# Autodesk Inventor assembly: blocker
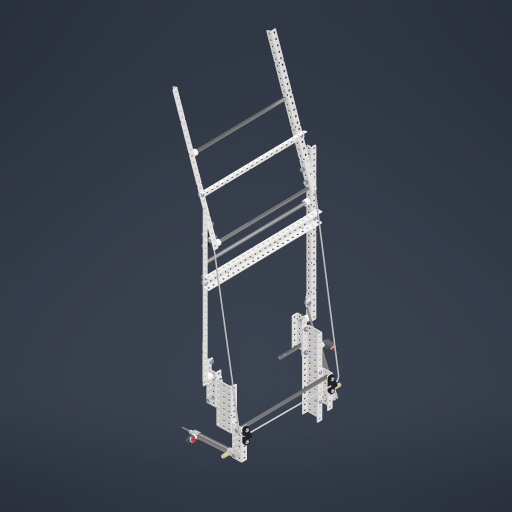
[picture p0: Inventor's stored thumbnail of the model, 512x512]
Saved by Autodesk Inventor 2024 (Build 280153000, 153)
## iProperties
Created: 2024-01-04
Part Number: blocker
Document SubType Name: Assembly
Designer: macbook
Author: macbook
## Documents named in this file (39)
- \\Mac\Home\Desktop\code\1599V-VRC\Cad\Assembly\v4\blocker.iam
- \\Mac\Home\Desktop\code\1599V-VRC\Cad\Assembly\v4\puncher.iam
- \\Mac\Home\Desktop\code\1599V-VRC\Cad\Structure\C Channel\Aluminum 1x3x1\Alu C 1x3x1x15.ipt
- \\Mac\Home\Desktop\code\1599V-VRC\Cad\Structure\C Channel\Aluminum 1x2x1\Alu C 1x2x1x6.ipt
- \\Mac\Home\Desktop\code\1599V-VRC\Cad\Motion\Pneumatics\Double Acting Piston.iam
- \\Mac\Home\Desktop\code\1599V-VRC\Cad\Structure\Standoff\Standoff 2.00.ipt
- \\Mac\Home\Desktop\code\1599V-VRC\Cad\Structure\Standoff.ipt
- \\Mac\Home\Desktop\code\1599V-VRC\Cad\Structure\C Channel\Aluminum 1x3x1\Alu C 1x3x1x8.ipt
- \\Mac\Home\Desktop\code\1599V-VRC\Cad\Structure\Standoff\Standoff 3.00.ipt
- \\Mac\Home\Desktop\code\1599V-VRC\Cad\Structure\Standoff\Standoff 6.00.ipt
- \\Mac\Home\Desktop\code\1599V-VRC\Cad\Motion\Spacers\Spacer Nylon .313 OD\NSpacer .313 OD x .125.ipt
- \\Mac\Home\Desktop\code\1599V-VRC\Cad\Motion\Spacers\Spacer Nylon .313 OD.ipt
- \\Mac\Home\Desktop\code\1599V-VRC\Cad\Structure\Angle\Aluminum\1x1\Alu Angle 1x1x30.ipt
- \\Mac\Home\Desktop\code\1599V-VRC\Cad\Motion\Spacers\Washer Teflon\TWasher .375 OD x .06250.ipt
- \\Mac\Home\Desktop\code\1599V-VRC\Cad\Motion\Spacers\Washer Teflon.ipt
- \\Mac\Home\Desktop\code\1599V-VRC\Cad\Structure\Angle\Aluminum\1x1\Alu Angle 1x1x1.ipt
- \\Mac\Home\Desktop\code\1599V-VRC\Cad\Structure\Hardware\Nut Nylock.ipt
- \\Mac\Home\Desktop\code\1599V-VRC\Cad\Structure\Angle\Aluminum\1x1\Alu Angle 1x1x25.ipt
- \\Mac\Home\Desktop\code\1599V-VRC\Cad\Motion\Shaft LS\Bearing Flat.ipt
- \\Mac\Home\Desktop\code\1599V-VRC\Cad\Structure\Hardware\Screw Steel - Star\SScrew Star Smooth .500.ipt
- \\Mac\Home\Desktop\code\1599V-VRC\Cad\Structure\Hardware\Screw Steel - Star.ipt
- \\Mac\Home\Desktop\code\1599V-VRC\Cad\Structure\Hardware\Nut Keps.ipt
- \\Mac\Home\Desktop\code\1599V-VRC\Cad\Motion\Shaft HS\HS Pillow Bearing Block.ipt
- \\Mac\Home\Desktop\code\1599V-VRC\Cad\Structure\Hardware\Screw Steel - Star\SScrew Star Smooth .375.ipt
- \\Mac\Home\Desktop\code\1599V-VRC\Cad\Motion\Pneumatics\Fitting for Cylinders.ipt
- \\Mac\Home\Desktop\code\1599V-VRC\Cad\Motion\Spacers\Spacer Nylon .500 OD\NSpacer White .500 OD x .500.ipt
- \\Mac\Home\Desktop\code\1599V-VRC\Cad\Motion\Spacers\Spacer Nylon .500 OD.ipt
- \\Mac\Home\Desktop\code\1599V-VRC\Cad\Structure\Hardware\Screw Steel - Star\SScrew Star Smooth .290.ipt
- \\Mac\Home\Desktop\code\1599V-VRC\Cad\Structure\Hardware\Screw Steel - Star\SScrew Star Smooth .875.ipt
- \\Mac\Home\Desktop\code\1599V-VRC\Cad\Motion\Insert Circle.ipt
- \\Mac\Home\Desktop\code\1599V-VRC\Cad\Structure\C Channel\Aluminum 1x2x1\Alu C 1x2x1x23.ipt
- \\Mac\Home\Desktop\code\1599V-VRC\Cad\Motion\Spacers\Spacer Nylon .313 OD\NSpacer .313 OD x .375.ipt
- \\Mac\Home\Desktop\code\1599V-VRC\Cad\Motion\Spacers\Spacer Nylon .500 OD\NSpacer White .500 OD x .375.ipt
- \\Mac\Home\Desktop\code\1599V-VRC\Cad\Structure\Angle\Aluminum\1x1\Alu Angle 1x1x21.ipt
- \\Mac\Home\Desktop\code\1599V-VRC\Cad\Structure\Standoff\Standoff 4.00.ipt
- \\Mac\Home\Desktop\code\1599V-VRC\Cad\Structure\Hardware\Nut Hex.ipt
- \\Mac\Home\Desktop\code\1599V-VRC\Cad\Structure\Hardware\Screw Steel - Star\SScrew Star Smooth .625.ipt
- \\Mac\Home\Desktop\code\1599V-VRC\Cad\Assembly\v4\blockerstring.ipt
- \\Mac\Home\Desktop\code\1599V-VRC\Cad\Motion\Pneumatics\Elbow Fitting\Elbow Fitting.ipt
## Components (132 placed, 33 different names)
1. puncher:1 [sub-assembly] — Insert:12, Insert:13, Insert:17, Insert:18
2. Alu C 1x3x1x15:1 — Insert:2, Insert:3, Insert:81, Insert:82, Insert:83, Insert:115, Insert:116, Insert:118
3. Alu C 1x2x1x6:1 — Insert:2, Insert:3, Insert:10, Insert:11, Insert:59, Insert:60, Insert:61, Insert:62, Insert:107, Insert:156
4. Alu C 1x2x1x6:4 — Insert:115, Insert:116, Insert:117
5. Standoff 2.00:1 — Insert:11, Insert:18
6. Standoff 2.00:2 — Insert:10, Insert:17
7. Standoff 2.00:3 — Insert:13, Insert:20
8. Standoff 2.00:4 — Insert:12, Insert:19
9. Alu C 1x2x1x6:2 — Insert:19, Insert:20, Insert:21, Insert:22, Insert:68, Insert:69, Insert:74, Insert:75, Insert:78, Insert:154
10. Alu C 1x2x1x6:3 — Insert:32, Insert:38, Insert:39, Insert:51, Insert:52, Insert:70, Insert:71, Insert:72, Insert:73, Insert:97, Insert:119, Insert:120
11. Alu C 1x3x1x8:1 — Insert:21, Insert:22, Insert:38, Insert:39, Insert:85, Insert:86, Insert:87, Insert:88
12. Standoff 3.00:5 — Insert:24
13. Standoff 6.00:6 — Insert:24
14. Alu Angle 1x1x30:1 — Insert:41, Insert:45, Insert:46, Insert:80, Insert:121, Insert:122, Insert:138, Insert:150, Insert:153, Insert:172, Insert:176, Insert:186, Insert:187
15. TWasher .375 OD x .06250:1 — Insert:32, Insert:40
16. Double Acting Piston:5 [sub-assembly] — Insert:40, Angle:1, Insert:76, Insert:96, Insert:98, Insert:188
17. Alu Angle 1x1x1:1 — Insert:41, Angle:1, Insert:42, Flush:1, Insert:158
18. Nut Nylock:1 — Insert:42
19. Alu Angle 1x1x25:1 — Insert:140, Angle:2, Angle:3, Insert:147, Insert:169, Insert:174, Insert:175, Insert:178, Insert:179, Insert:180
20. Bearing Flat:1 — Insert:45, Insert:46, Insert:47, Insert:48
21. SScrew Star Smooth .500:1 — Insert:47
22. SScrew Star Smooth .500:2 — Insert:48
23. HS Pillow Bearing Block:1 — Insert:51, Insert:52, Insert:89, Insert:93
24. HS Pillow Bearing Block:2 — Insert:91, Insert:92, Rotational:1
25. SScrew Star Smooth .375:3 — Insert:61
26. SScrew Star Smooth .375:4
27. SScrew Star Smooth .375:5 — Insert:60
28. SScrew Star Smooth .375:6 — Insert:62
29. SScrew Star Smooth .375:7 — Insert:59
30. SScrew Star Smooth .375:8
31. SScrew Star Smooth .375:10
32. SScrew Star Smooth .375:11
33. SScrew Star Smooth .375:12 — Insert:69
34. SScrew Star Smooth .375:13 — Insert:68
35. SScrew Star Smooth .375:14 — Insert:70
36. SScrew Star Smooth .375:17 — Insert:71
37. SScrew Star Smooth .375:18 — Insert:73
38. SScrew Star Smooth .375:19 — Insert:72
39. SScrew Star Smooth .375:20 — Insert:75
40. SScrew Star Smooth .375:21 — Insert:74
41. Fitting for Cylinders:1 — Insert:76
42. NSpacer White .500 OD x .500:1 — Insert:78, Insert:79
43. TWasher .375 OD x .06250:2 — Insert:79, Insert:80
44. Nut Nylock:2 — Insert:81
45. Nut Nylock:3 — Insert:82
46. Nut Nylock:5 — Insert:83
47. Nut Nylock:7 — Insert:86
48. Nut Nylock:8 — Insert:85
49. Nut Nylock:9 — Insert:88
50. Nut Nylock:10 — Insert:87
51. Nut Nylock:11 — Insert:89
52. Nut Nylock:13 — Insert:91
53. Nut Nylock:14 — Insert:92
54. Nut Nylock:15 — Insert:93
55. SScrew Star Smooth .875:23 — Insert:96
56. Nut Nylock:16 — Insert:97
57. Insert Circle:1 — Insert:98
58. TWasher .375 OD x .06250:3
59. Double Acting Piston:6 [sub-assembly] — Insert:189
60. Fitting for Cylinders:3
61. SScrew Star Smooth .875:24
62. Insert Circle:2
63. Nut Nylock:17
64. NSpacer White .500 OD x .500:2 — Insert:107, Insert:108
65. Alu Angle 1x1x30:2 — Insert:111, Insert:112, Insert:114, Insert:125, Insert:126, Insert:127, Insert:128, Insert:135, Insert:155, Insert:161, Insert:183, Insert:184, Insert:185
66. NSpacer .313 OD x .125:4 — Insert:108
67. Alu C 1x2x1x23:1 — Insert:111, Insert:112, Insert:159, Insert:160, Insert:170, Insert:171
68. Alu Angle 1x1x1:2 — Insert:114, Flush:1, Insert:157
69. Nut Nylock:18
70. SScrew Star Smooth .375:25 — Insert:117
71. Nut Nylock:19 — Insert:118
72. NSpacer .313 OD x .125:5 — Insert:119
73. SScrew Star Smooth .290:26 — Insert:120
74. Nut Keps:3 — Insert:122
75. Nut Keps:4 — Insert:121
76. Bearing Flat:2 — Insert:125, Insert:126
77. SScrew Star Smooth .500:27
78. SScrew Star Smooth .500:28
79. Nut Keps:5 — Insert:127
80. Nut Keps:6 — Insert:128
81. Alu Angle 1x1x25:2 — Insert:136, Insert:144, Angle:2, Insert:162, Insert:163, Insert:165, Insert:167, Insert:181, Insert:182
82. NSpacer .313 OD x .375:6 — Insert:134, Insert:135
83. TWasher .375 OD x .06250:4 — Insert:134, Insert:136
84. NSpacer .313 OD x .375:7 — Insert:138
85. TWasher .375 OD x .06250:5
86. Standoff 3.00:11 — Insert:141, Insert:142
87. Standoff 6.00:12 — Insert:142
88. NSpacer White .500 OD x .375:3 — Insert:140, Insert:141
89. Alu Angle 1x1x21:1 — Insert:144, Angle:3, Insert:166, Insert:173
90. Standoff 3.00:13
91. Standoff 6.00:14
92. NSpacer White .500 OD x .375:4 — Insert:147
93. Standoff 4.00:15 — Insert:151
94. Standoff 6.00:16 — Insert:150
95. NSpacer White .500 OD x .375:5 — Insert:151
96. SScrew Star Smooth .875:29 — Insert:153
97. Nut Nylock:20 — Insert:154
98. SScrew Star Smooth .875:30 — Insert:155
99. Nut Nylock:21 — Insert:156
100. Nut Hex:1 — Insert:157
101. Nut Hex:2 — Insert:158
102. SScrew Star Smooth .375:31 — Insert:159
103. SScrew Star Smooth .375:32 — Insert:160
104. SScrew Star Smooth .375:33 — Insert:161
105. SScrew Star Smooth .375:34 — Insert:162
106. NSpacer .313 OD x .375:9 — Insert:163, Insert:164
107. SScrew Star Smooth .625:35 — Insert:164
108. Nut Nylock:22 — Insert:165
109. SScrew Star Smooth .375:36 — Insert:166
110. SScrew Star Smooth .375:37 — Insert:167
111. NSpacer .313 OD x .375:10 — Insert:169
112. SScrew Star Smooth .625:38
113. SScrew Star Smooth .375:39 — Insert:170
114. SScrew Star Smooth .375:40 — Insert:171
115. SScrew Star Smooth .375:41 — Insert:172
116. SScrew Star Smooth .375:42 — Insert:173
117. SScrew Star Smooth .375:43 — Insert:174
118. SScrew Star Smooth .375:44 — Insert:175
119. SScrew Star Smooth .875:45 — Insert:176
120. Nut Nylock:23 — Insert:178
121. Nut Nylock:24 — Insert:179
122. Nut Nylock:25 — Insert:180
123. Nut Nylock:26 — Insert:181
124. Nut Nylock:27 — Insert:182
125. SScrew Star Smooth .875:47 — Insert:183
126. Nut Nylock:28 — Insert:184
127. Nut Nylock:29 — Insert:185
128. Nut Nylock:30 — Insert:186
129. Nut Nylock:31 — Insert:187
130. blockerstring:2 — Rotational:1
131. Elbow Fitting:1 — Insert:188
132. Elbow Fitting:2 — Insert:189
## Relationships (147: Insert 142, Angle 3, Flush 1, RevoluteJoint 1)
- Insert:2: Alu C 1x3x1x15:1 ↔ Alu C 1x2x1x6:1
- Insert:3: Alu C 1x3x1x15:1 ↔ Alu C 1x2x1x6:1
- Insert:10: Alu C 1x2x1x6:1 ↔ Standoff 2.00:2
- Insert:11: Alu C 1x2x1x6:1 ↔ Standoff 2.00:1
- Insert:12: puncher:1 ↔ Standoff 2.00:4
- Insert:13: puncher:1 ↔ Standoff 2.00:3
- Insert:17: puncher:1 ↔ Standoff 2.00:2
- Insert:18: puncher:1 ↔ Standoff 2.00:1
- Insert:19: Standoff 2.00:4 ↔ Alu C 1x2x1x6:2
- Insert:20: Standoff 2.00:3 ↔ Alu C 1x2x1x6:2
- Insert:21: Alu C 1x2x1x6:2 ↔ Alu C 1x3x1x8:1
- Insert:22: Alu C 1x2x1x6:2 ↔ Alu C 1x3x1x8:1
- Insert:24: Standoff 3.00:5 ↔ Standoff 6.00:6
- [Insert]: Alu C 1x2x1x6:4 ↔ Standoff 3.00:5
- Insert:32: Alu C 1x2x1x6:3 ↔ TWasher .375 OD x .06250:1
- Insert:38: Alu C 1x2x1x6:3 ↔ Alu C 1x3x1x8:1
- Insert:39: Alu C 1x2x1x6:3 ↔ Alu C 1x3x1x8:1
- Insert:40: TWasher .375 OD x .06250:1 ↔ Double Acting Piston:5
- Insert:41: Alu Angle 1x1x30:1 ↔ Alu Angle 1x1x1:1
- Angle:1 (0 deg): Double Acting Piston:5 ↔ Alu Angle 1x1x1:1
- Insert:42: Alu Angle 1x1x1:1 ↔ Nut Nylock:1
- Insert:45: Alu Angle 1x1x30:1 ↔ Bearing Flat:1
- Insert:46: Alu Angle 1x1x30:1 ↔ Bearing Flat:1
- Insert:47: Bearing Flat:1 ↔ SScrew Star Smooth .500:1
- Insert:48: Bearing Flat:1 ↔ SScrew Star Smooth .500:2
- Insert:51: Alu C 1x2x1x6:3 ↔ HS Pillow Bearing Block:1
- Insert:52: Alu C 1x2x1x6:3 ↔ HS Pillow Bearing Block:1
- [Insert]: Alu C 1x2x1x6:4 ↔ HS Pillow Bearing Block:2
- [Insert]: Alu C 1x2x1x6:4 ↔ HS Pillow Bearing Block:2
- Insert:59: Alu C 1x2x1x6:1 ↔ SScrew Star Smooth .375:7
- Insert:60: Alu C 1x2x1x6:1 ↔ SScrew Star Smooth .375:5
- Insert:61: Alu C 1x2x1x6:1 ↔ SScrew Star Smooth .375:3
- Insert:62: Alu C 1x2x1x6:1 ↔ SScrew Star Smooth .375:6
- [Insert]: Alu C 1x2x1x6:4 ↔ SScrew Star Smooth .375:4
- [Insert]: Alu C 1x2x1x6:4 ↔ SScrew Star Smooth .375:8
- [Insert]: Alu C 1x2x1x6:4 ↔ SScrew Star Smooth .375:11
- [Insert]: Alu C 1x2x1x6:4 ↔ SScrew Star Smooth .375:10
- Insert:68: Alu C 1x2x1x6:2 ↔ SScrew Star Smooth .375:13
- Insert:69: Alu C 1x2x1x6:2 ↔ SScrew Star Smooth .375:12
- Insert:70: Alu C 1x2x1x6:3 ↔ SScrew Star Smooth .375:14
- Insert:71: Alu C 1x2x1x6:3 ↔ SScrew Star Smooth .375:17
- Insert:72: Alu C 1x2x1x6:3 ↔ SScrew Star Smooth .375:19
- Insert:73: Alu C 1x2x1x6:3 ↔ SScrew Star Smooth .375:18
- Insert:74: Alu C 1x2x1x6:2 ↔ SScrew Star Smooth .375:21
- Insert:75: Alu C 1x2x1x6:2 ↔ SScrew Star Smooth .375:20
- Insert:76: Double Acting Piston:5 ↔ Fitting for Cylinders:1
- Insert:78: Alu C 1x2x1x6:2 ↔ NSpacer White .500 OD x .500:1
- Insert:79: NSpacer White .500 OD x .500:1 ↔ TWasher .375 OD x .06250:2
- Insert:80: Alu Angle 1x1x30:1 ↔ TWasher .375 OD x .06250:2
- Insert:81: Alu C 1x3x1x15:1 ↔ Nut Nylock:2
- Insert:82: Alu C 1x3x1x15:1 ↔ Nut Nylock:3
- Insert:83: Alu C 1x3x1x15:1 ↔ Nut Nylock:5
- Insert:85: Alu C 1x3x1x8:1 ↔ Nut Nylock:8
- Insert:86: Alu C 1x3x1x8:1 ↔ Nut Nylock:7
- Insert:87: Alu C 1x3x1x8:1 ↔ Nut Nylock:10
- Insert:88: Alu C 1x3x1x8:1 ↔ Nut Nylock:9
- Insert:89: HS Pillow Bearing Block:1 ↔ Nut Nylock:11
- Insert:91: HS Pillow Bearing Block:2 ↔ Nut Nylock:13
- Insert:92: HS Pillow Bearing Block:2 ↔ Nut Nylock:14
- Insert:93: HS Pillow Bearing Block:1 ↔ Nut Nylock:15
- Insert:96: Double Acting Piston:5 ↔ SScrew Star Smooth .875:23
- Insert:97: Alu C 1x2x1x6:3 ↔ Nut Nylock:16
- Insert:98: Double Acting Piston:5 ↔ Insert Circle:1
- [Insert]: TWasher .375 OD x .06250:3 ↔ Double Acting Piston:6
- [Insert]: Double Acting Piston:6 ↔ Fitting for Cylinders:3
- [Insert]: Double Acting Piston:6 ↔ SScrew Star Smooth .875:24
- [Insert]: Double Acting Piston:6 ↔ Insert Circle:2
- [Insert]: Alu C 1x2x1x6:4 ↔ TWasher .375 OD x .06250:3
- [Insert]: Alu C 1x2x1x6:4 ↔ Nut Nylock:17
- Insert:107: Alu C 1x2x1x6:1 ↔ NSpacer White .500 OD x .500:2
- Insert:108: NSpacer White .500 OD x .500:2 ↔ NSpacer .313 OD x .125:4
- [Insert]: Alu Angle 1x1x30:1 ↔ Alu C 1x2x1x23:1
- [Insert]: Alu Angle 1x1x30:1 ↔ Alu C 1x2x1x23:1
- Insert:111: Alu Angle 1x1x30:2 ↔ Alu C 1x2x1x23:1
- Insert:112: Alu Angle 1x1x30:2 ↔ Alu C 1x2x1x23:1
- [Insert]: Alu Angle 1x1x1:2 ↔ Nut Nylock:18
- Insert:114: Alu Angle 1x1x30:2 ↔ Alu Angle 1x1x1:2
- Insert:115: Alu C 1x3x1x15:1 ↔ Alu C 1x2x1x6:4
- Insert:116: Alu C 1x3x1x15:1 ↔ Alu C 1x2x1x6:4
- Insert:117: Alu C 1x2x1x6:4 ↔ SScrew Star Smooth .375:25
- Insert:118: Alu C 1x3x1x15:1 ↔ Nut Nylock:19
- Insert:119: Alu C 1x2x1x6:3 ↔ NSpacer .313 OD x .125:5
- Insert:120: Alu C 1x2x1x6:3 ↔ SScrew Star Smooth .290:26
- Flush:1: Alu Angle 1x1x1:1 ↔ Alu Angle 1x1x1:2
- Insert:121: Alu Angle 1x1x30:1 ↔ Nut Keps:4
- Insert:122: Alu Angle 1x1x30:1 ↔ Nut Keps:3
- [Insert]: Bearing Flat:2 ↔ SScrew Star Smooth .500:27
- [Insert]: Bearing Flat:2 ↔ SScrew Star Smooth .500:28
- Insert:125: Alu Angle 1x1x30:2 ↔ Bearing Flat:2
- Insert:126: Alu Angle 1x1x30:2 ↔ Bearing Flat:2
- Insert:127: Alu Angle 1x1x30:2 ↔ Nut Keps:5
- Insert:128: Alu Angle 1x1x30:2 ↔ Nut Keps:6
- Insert:134: NSpacer .313 OD x .375:6 ↔ TWasher .375 OD x .06250:4
- Insert:135: Alu Angle 1x1x30:2 ↔ NSpacer .313 OD x .375:6
- Insert:136: Alu Angle 1x1x25:2 ↔ TWasher .375 OD x .06250:4
- [Insert]: NSpacer .313 OD x .375:7 ↔ TWasher .375 OD x .06250:5
- Insert:138: Alu Angle 1x1x30:1 ↔ NSpacer .313 OD x .375:7
- Insert:140: Alu Angle 1x1x25:1 ↔ NSpacer White .500 OD x .375:3
- Insert:141: Standoff 3.00:11 ↔ NSpacer White .500 OD x .375:3
- Insert:142: Standoff 3.00:11 ↔ Standoff 6.00:12
- [Insert]: Alu Angle 1x1x25:1 ↔ Alu Angle 1x1x21:1
- Insert:144: Alu Angle 1x1x25:2 ↔ Alu Angle 1x1x21:1
- Angle:2 (0 deg): Alu Angle 1x1x25:1 ↔ Alu Angle 1x1x25:2
- Angle:3 (90 deg): Alu Angle 1x1x25:1 ↔ Alu Angle 1x1x21:1
- [Insert]: Standoff 3.00:13 ↔ NSpacer White .500 OD x .375:4
- [Insert]: Standoff 3.00:13 ↔ Standoff 6.00:14
- Insert:147: Alu Angle 1x1x25:1 ↔ NSpacer White .500 OD x .375:4
- [Insert]: Standoff 4.00:15 ↔ Standoff 6.00:16
- Insert:150: Alu Angle 1x1x30:1 ↔ Standoff 6.00:16
- Insert:151: Standoff 4.00:15 ↔ NSpacer White .500 OD x .375:5
- Insert:153: Alu Angle 1x1x30:1 ↔ SScrew Star Smooth .875:29
- Insert:154: Alu C 1x2x1x6:2 ↔ Nut Nylock:20
- Insert:155: Alu Angle 1x1x30:2 ↔ SScrew Star Smooth .875:30
- Insert:156: Alu C 1x2x1x6:1 ↔ Nut Nylock:21
- Insert:157: Alu Angle 1x1x1:2 ↔ Nut Hex:1
- Insert:158: Alu Angle 1x1x1:1 ↔ Nut Hex:2
- Insert:159: Alu C 1x2x1x23:1 ↔ SScrew Star Smooth .375:31
- Insert:160: Alu C 1x2x1x23:1 ↔ SScrew Star Smooth .375:32
- Insert:161: Alu Angle 1x1x30:2 ↔ SScrew Star Smooth .375:33
- Insert:162: Alu Angle 1x1x25:2 ↔ SScrew Star Smooth .375:34
- Insert:163: Alu Angle 1x1x25:2 ↔ NSpacer .313 OD x .375:9
- Insert:164: NSpacer .313 OD x .375:9 ↔ SScrew Star Smooth .625:35
- Insert:165: Alu Angle 1x1x25:2 ↔ Nut Nylock:22
- Insert:166: Alu Angle 1x1x21:1 ↔ SScrew Star Smooth .375:36
- Insert:167: Alu Angle 1x1x25:2 ↔ SScrew Star Smooth .375:37
- [Insert]: NSpacer .313 OD x .375:10 ↔ SScrew Star Smooth .625:38
- Insert:169: Alu Angle 1x1x25:1 ↔ NSpacer .313 OD x .375:10
- Insert:170: Alu C 1x2x1x23:1 ↔ SScrew Star Smooth .375:39
- Insert:171: Alu C 1x2x1x23:1 ↔ SScrew Star Smooth .375:40
- Insert:172: Alu Angle 1x1x30:1 ↔ SScrew Star Smooth .375:41
- Insert:173: Alu Angle 1x1x21:1 ↔ SScrew Star Smooth .375:42
- Insert:174: Alu Angle 1x1x25:1 ↔ SScrew Star Smooth .375:43
- Insert:175: Alu Angle 1x1x25:1 ↔ SScrew Star Smooth .375:44
- Insert:176: Alu Angle 1x1x30:1 ↔ SScrew Star Smooth .875:45
- Insert:178: Alu Angle 1x1x25:1 ↔ Nut Nylock:23
- Insert:179: Alu Angle 1x1x25:1 ↔ Nut Nylock:24
- Insert:180: Alu Angle 1x1x25:1 ↔ Nut Nylock:25
- Insert:181: Alu Angle 1x1x25:2 ↔ Nut Nylock:26
- Insert:182: Alu Angle 1x1x25:2 ↔ Nut Nylock:27
- Insert:183: Alu Angle 1x1x30:2 ↔ SScrew Star Smooth .875:47
- Insert:184: Alu Angle 1x1x30:2 ↔ Nut Nylock:28
- Insert:185: Alu Angle 1x1x30:2 ↔ Nut Nylock:29
- Insert:186: Alu Angle 1x1x30:1 ↔ Nut Nylock:30
- Insert:187: Alu Angle 1x1x30:1 ↔ Nut Nylock:31
- Rotational:1 [RevoluteJoint] (-114.3 mm): HS Pillow Bearing Block:2 ↔ blockerstring:2
- Insert:188: Double Acting Piston:5 ↔ Elbow Fitting:1
- Insert:189: Double Acting Piston:6 ↔ Elbow Fitting:2
## Named parameters: d124_d121 = 0 mm, d125_d123 = 0 mm, d126_d100 = 0 mm, d128_d49 = 0 mm, d139_d54 = 0 mm, d150_d61 = 0 mm, d151_d60 = 0 mm, d164_d161 = 0 mm, d176_d170 = 0 mm, d177_d171 = 0 mm, d180_d171 = 0 mm, d199_d195 = 0 mm
